# Autodesk Inventor assembly: mount_assembly
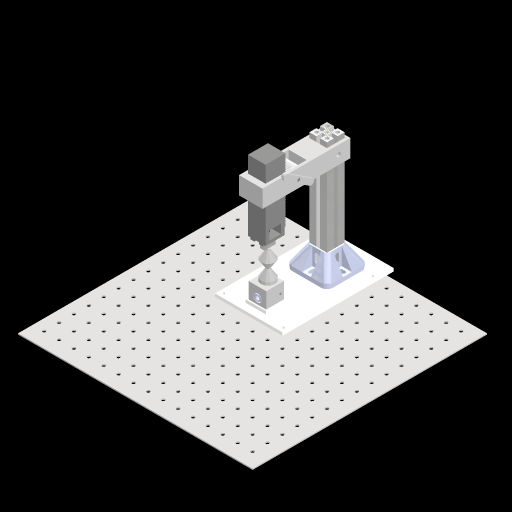
[picture p0: Inventor's stored thumbnail of the model, 512x512]
Saved by Autodesk Inventor 2023 (Build 270158000, 158)
## iProperties
Created: 2024-07-03
Part Number: mount_assembly
Document SubType Name: Assembly
Designer: OMS55
Author: OMS55
## Documents named in this file (16)
- C:\Users\OMS55\OneDrive\Documents\성균관대학교\LAB\성균관대 최혁렬 교수님\testbed_mount\mount_assembly.iam
- C:\Users\OMS55\OneDrive\Documents\성균관대학교\LAB\성균관대 최혁렬 교수님\testbed_mount\mounting_board.ipt
- C:\Users\OMS55\OneDrive\Documents\성균관대학교\LAB\성균관대 최혁렬 교수님\testbed_mount\mounting_board_printed.ipt
- C:\Users\OMS55\OneDrive\Documents\성균관대학교\LAB\성균관대 최혁렬 교수님\testbed_mount\3030_base.ipt
- C:\Users\OMS55\OneDrive\Documents\성균관대학교\LAB\성균관대 최혁렬 교수님\testbed_mount\3030column.ipt
- C:\Users\OMS55\OneDrive\Documents\성균관대학교\LAB\성균관대 최혁렬 교수님\testbed_mount\lever_support.ipt
- C:\Users\OMS55\OneDrive\Documents\성균관대학교\LAB\성균관대 최혁렬 교수님\testbed_mount\valve_mount.ipt
- C:\Users\OMS55\OneDrive\Documents\성균관대학교\LAB\성균관대 최혁렬 교수님\testbed_mount\GPL 06M5(L)(3D).iam
- C:\Users\OMS55\OneDrive\Documents\성균관대학교\LAB\성균관대 최혁렬 교수님\testbed_mount\valve_mount_pin.ipt
- C:\Users\OMS55\OneDrive\Documents\성균관대학교\LAB\성균관대 최혁렬 교수님\testbed_mount\rp_lever.ipt
- C:\Users\OMS55\OneDrive\Documents\성균관대학교\LAB\성균관대 최혁렬 교수님\testbed_mount\cell_pin.ipt
- C:\Users\OMS55\OneDrive\Documents\성균관대학교\LAB\성균관대 최혁렬 교수님\testbed_mount\loadcell.ipt
- C:\Users\OMS55\OneDrive\Documents\성균관대학교\LAB\성균관대 최혁렬 교수님\testbed_mount\finger.ipt
- C:\Users\OMS55\OneDrive\Documents\성균관대학교\LAB\성균관대 최혁렬 교수님\testbed_mount\lever_handle.ipt
- C:\Users\OMS55\OneDrive\Documents\성균관대학교\LAB\성균관대 최혁렬 교수님\testbed_mount\pinion_gear.ipt
- C:\Users\OMS55\OneDrive\Documents\성균관대학교\LAB\성균관대 최혁렬 교수님\testbed_mount\rack_gear.ipt
## Components (15 placed, 15 different names)
1. mounting_board:1 — 메이트:1, 메이트:2, 메이트:3
2. mounting_board_printed:1 — 메이트:1, 메이트:2, 메이트:3, 메이트:4, 메이트:5, 각도:1, 메이트:20, 메이트:21, 메이트:22
3. 3030_base:1 — 메이트:6, 메이트:7, 메이트:8, 각도:1
4. 3030column:1 — 메이트:4, 메이트:5, 메이트:6, 메이트:7, 메이트:8, 메이트:9, 메이트:10
5. lever_support:1 — 메이트:9, 메이트:10, 메이트:28, 메이트:29, 메이트:30, 메이트:31
6. GPL 06M5(L)(3D):1 [sub-assembly] — 메이트:23, 플러쉬:2, 각도:2, 메이트:26
7. valve_mount:1 — 메이트:20, 메이트:21, 메이트:22, 메이트:23, 플러쉬:2, 각도:2, 메이트:24, 메이트:25, 메이트:27
8. valve_mount_pin:1 — 메이트:24, 메이트:25
9. finger:1 — 메이트:26, 메이트:27
10. cell_pin:1 — 메이트:38, 메이트:39
11. lever_handle:1 — 플러쉬:3, 메이트:34, 메이트:35
12. loadcell:1 — 메이트:36, 각도:3, 메이트:37
13. pinion_gear:1 — 메이트:30, 메이트:31, 메이트:32, 메이트:33
14. rack_gear:1 — 메이트:28, 메이트:29, 메이트:36, 각도:3, 메이트:37, 메이트:38, 메이트:39
15. rp_lever:1 — 메이트:32, 메이트:33, 플러쉬:3, 메이트:34, 메이트:35
## Relationships (35: Mate 30, Angle 3, Flush 2)
- 메이트:1 [Mate]: mounting_board:1 ↔ mounting_board_printed:1
- 메이트:2 [Mate]: mounting_board:1 ↔ mounting_board_printed:1
- 메이트:3 [Mate]: mounting_board:1 ↔ mounting_board_printed:1
- 메이트:4 [Mate]: mounting_board_printed:1 ↔ 3030column:1
- 메이트:5 [Mate]: mounting_board_printed:1 ↔ 3030column:1
- 메이트:6 [Mate]: 3030_base:1 ↔ 3030column:1
- 메이트:7 [Mate]: 3030_base:1 ↔ 3030column:1
- 메이트:8 [Mate]: 3030_base:1 ↔ 3030column:1
- 각도:1 [Angle] (0 deg): mounting_board_printed:1 ↔ 3030_base:1
- 메이트:9 [Mate]: 3030column:1 ↔ lever_support:1
- 메이트:10 [Mate]: 3030column:1 ↔ lever_support:1
- 메이트:20 [Mate]: mounting_board_printed:1 ↔ valve_mount:1
- 메이트:21 [Mate]: mounting_board_printed:1 ↔ valve_mount:1
- 메이트:22 [Mate]: mounting_board_printed:1 ↔ valve_mount:1
- 메이트:23 [Mate]: GPL 06M5(L)(3D):1 ↔ valve_mount:1
- 플러쉬:2 [Flush]: GPL 06M5(L)(3D):1 ↔ valve_mount:1
- 각도:2 [Angle] (0 deg): GPL 06M5(L)(3D):1 ↔ valve_mount:1
- 메이트:24 [Mate]: valve_mount:1 ↔ valve_mount_pin:1
- 메이트:25 [Mate]: valve_mount:1 ↔ valve_mount_pin:1
- 메이트:26 [Mate]: GPL 06M5(L)(3D):1 ↔ finger:1
- 메이트:27 [Mate]: valve_mount:1 ↔ finger:1
- 메이트:28 [Mate]: lever_support:1 ↔ rack_gear:1
- 메이트:29 [Mate]: lever_support:1 ↔ rack_gear:1
- 메이트:30 [Mate]: lever_support:1 ↔ pinion_gear:1
- 메이트:31 [Mate]: lever_support:1 ↔ pinion_gear:1
- 메이트:32 [Mate]: pinion_gear:1 ↔ rp_lever:1
- 메이트:33 [Mate]: pinion_gear:1 ↔ rp_lever:1
- 플러쉬:3 [Flush]: lever_handle:1 ↔ rp_lever:1
- 메이트:34 [Mate]: lever_handle:1 ↔ rp_lever:1
- 메이트:35 [Mate]: lever_handle:1 ↔ rp_lever:1
- 메이트:36 [Mate]: loadcell:1 ↔ rack_gear:1
- 각도:3 [Angle] (0 deg): loadcell:1 ↔ rack_gear:1
- 메이트:37 [Mate]: loadcell:1 ↔ rack_gear:1
- 메이트:38 [Mate]: cell_pin:1 ↔ rack_gear:1
- 메이트:39 [Mate]: cell_pin:1 ↔ rack_gear:1
